# Autodesk Inventor assembly: AMR_Transm2
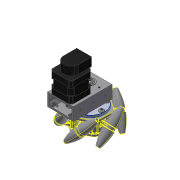
[picture p0: Inventor's stored thumbnail of the model, 180x180]
Saved by Autodesk Inventor 2018 (Build 220112000, 112)
## iProperties
Created: 2019-08-30
Part Number: AMR_Transm2
Document SubType Name: Assembly
Designer: Clevo
Author: Clevo
## Documents named in this file (20)
- E:\Hardware_Accelerated_Robot\Hardware\AMR_Transm2.iam
- E:\Hardware_Accelerated_Robot\Hardware\nema-17-12.snapshot.1\Nema 17\Nema 17.ipt
- E:\Hardware_Accelerated_Robot\Hardware\CustomParts\Transmission_Case.ipt
- E:\Hardware_Accelerated_Robot\Hardware\Bearings\7804K136_STAINLESS STEEL BALL BEARING.ipt
- E:\Hardware_Accelerated_Robot\Hardware\Wheels\am-3026L 4HD Mecanum Left V3 With Screws.ipt
- E:\Hardware_Accelerated_Robot\Hardware\Wheels\am-0096a 500 Hex Hub r2.ipt
- E:\Hardware_Accelerated_Robot\Hardware\CustomParts\Axle.ipt
- E:\Hardware_Accelerated_Robot\Hardware\Bearings\7804K147_STAINLESS STEEL BALL BEARING.ipt
- E:\Hardware_Accelerated_Robot\Hardware\Screws\94500A231_TYPE 316 SS BUTTON-HEAD SOCKET CAP SCREW.ipt
- E:\Hardware_Accelerated_Robot\Hardware\Screws\96660A215_FLANGED BUTTON-HEAD SOCKET CAP SCREW.ipt
- E:\Hardware_Accelerated_Robot\Hardware\Pulleys\gt2-40-teeth-bore-8mm-belt-6mm-1.snapshot.1\GT2_40T_8_6.ipt
- E:\Hardware_Accelerated_Robot\Hardware\Pulleys\timing-pulley-gt2-20t-8mm-bore-1.snapshot.8\GT2_20T-sh8.ipt
- E:\Hardware_Accelerated_Robot\Hardware\Bearings\5905K348_STEEL NEEDLE-ROLLER BEARING.ipt
- E:\Hardware_Accelerated_Robot\Hardware\AMR_Transm\Design Accelerator\Synchronous Belts Transmission1.iam
- E:\Hardware_Accelerated_Robot\Hardware\CustomParts\Tensioner.ipt
- E:\Hardware_Accelerated_Robot\Hardware\Screws\92137A262_CLASS 10.9 ALLOY STEEL BUTTON-HEAD CAP SCREW.ipt
- E:\Hardware_Accelerated_Robot\Hardware\Wheels\am-2538 - 4 in mecanum left wheel.ipt
- E:\Hardware_Accelerated_Robot\Hardware\Wheels\am-2256 4 in HiGrip Wheel.ipt
- E:\Hardware_Accelerated_Robot\Hardware\CustomParts\Transmission_Case_ForPrint.ipt
- E:\Hardware_Accelerated_Robot\Hardware\Screws\91385A211_THREAD-LOCKING CUP POINT SET SCREW.ipt
## Components (25 placed, 19 different names)
1. Nema 17:1 — Mate:1, Mate:2, Mate:3, Mate:4, Mate:32
2. Transmission_Case:1 — Mate:1, Mate:2, Mate:3, Mate:5, Mate:10, Mate:11, Mate:12, Mate:13, Mate:34, Mate:35, Mate:36, Flush:4, Flush:5, Mate:49
3. 7804K136_STAINLESS STEEL BALL BEARING:1 — Mate:4, Mate:5, Mate:33
4. am-3026L 4HD Mecanum Left V3 With Screws:1 — Mate:6, Mate:7, Mate:8
5. am-0096a 500 Hex Hub r2:1 — Mate:6, Mate:7, Mate:8, Mate:9, Flush:1, Angle:1, Mate:14, Mate:15, Mate:16, Mate:17, Mate:18, Mate:19, Mate:20, Mate:21, Mate:22, Mate:23, Mate:24, Mate:25, Mate:40, Mate:41, Mate:42, Mate:43, Mate:44, Mate:45, Mate:47
6. Axle:1 — Mate:9, Flush:1, Angle:1, Mate:26, Mate:28, Mate:29, Mate:30, Mate:48
7. 7804K147_STAINLESS STEEL BALL BEARING:1 — Mate:10, Mate:13, Mate:26
8. 7804K147_STAINLESS STEEL BALL BEARING:2 — Mate:11, Mate:12, Mate:27
9. 94500A231_TYPE 316 SS BUTTON-HEAD SOCKET CAP SCREW:1 — Mate:16, Mate:21
10. 94500A231_TYPE 316 SS BUTTON-HEAD SOCKET CAP SCREW:2 — Mate:17, Mate:22
11. 94500A231_TYPE 316 SS BUTTON-HEAD SOCKET CAP SCREW:3 — Mate:15, Mate:23
12. 94500A231_TYPE 316 SS BUTTON-HEAD SOCKET CAP SCREW:4 — Mate:14, Mate:20
13. 94500A231_TYPE 316 SS BUTTON-HEAD SOCKET CAP SCREW:5 — Mate:19, Mate:24
14. 94500A231_TYPE 316 SS BUTTON-HEAD SOCKET CAP SCREW:6 — Mate:18, Mate:25
15. 96660A215_FLANGED BUTTON-HEAD SOCKET CAP SCREW:1 — Mate:28, Mate:29, Mate:27
16. GT2_40T_8_6:1 — Mate:30, Flush:2
17. GT2_20T-sh8:1 — Mate:32, Flush:2, Mate:33
18. 5905K348_STEEL NEEDLE-ROLLER BEARING:1 — Mate:34, Mate:37
19. Synchronous Belts Transmission:1 [sub-assembly]
20. Tensioner:1 — Mate:35, Mate:36, Mate:37, Mate:38, Mate:39
21. 92137A262_CLASS 10.9 ALLOY STEEL BUTTON-HEAD CAP SCREW:1 — Mate:38, Mate:39
22. am-2538 - 4 in mecanum left wheel:1 — Mate:40, Mate:41, Mate:42
23. am-2256 4 in HiGrip Wheel:1 — Mate:43, Mate:44, Mate:45
24. Transmission_Case_ForPrint:1 — Flush:4, Flush:5, Mate:49
25. 91385A211_THREAD-LOCKING CUP POINT SET SCREW:1 — Mate:47, Mate:48
## Relationships (52: Mate 47, Flush 4, Angle 1)
- Mate:1: Nema 17:1 ↔ Transmission_Case:1
- Mate:2: Nema 17:1 ↔ Transmission_Case:1
- Mate:3: Nema 17:1 ↔ Transmission_Case:1
- Mate:4: Nema 17:1 ↔ 7804K136_STAINLESS STEEL BALL BEARING:1
- Mate:5: Transmission_Case:1 ↔ 7804K136_STAINLESS STEEL BALL BEARING:1
- Mate:6: am-3026L 4HD Mecanum Left V3 With Screws:1 ↔ am-0096a 500 Hex Hub r2:1
- Mate:7: am-3026L 4HD Mecanum Left V3 With Screws:1 ↔ am-0096a 500 Hex Hub r2:1
- Mate:8: am-3026L 4HD Mecanum Left V3 With Screws:1 ↔ am-0096a 500 Hex Hub r2:1
- Mate:9: am-0096a 500 Hex Hub r2:1 ↔ Axle:1
- Flush:1: am-0096a 500 Hex Hub r2:1 ↔ Axle:1
- Angle:1 (0 deg): am-0096a 500 Hex Hub r2:1 ↔ Axle:1
- Mate:10: Transmission_Case:1 ↔ 7804K147_STAINLESS STEEL BALL BEARING:1
- Mate:11: Transmission_Case:1 ↔ 7804K147_STAINLESS STEEL BALL BEARING:2
- Mate:12: Transmission_Case:1 ↔ 7804K147_STAINLESS STEEL BALL BEARING:2
- Mate:13: Transmission_Case:1 ↔ 7804K147_STAINLESS STEEL BALL BEARING:1
- Mate:14: am-0096a 500 Hex Hub r2:1 ↔ 94500A231_TYPE 316 SS BUTTON-HEAD SOCKET CAP SCREW:4
- Mate:15: am-0096a 500 Hex Hub r2:1 ↔ 94500A231_TYPE 316 SS BUTTON-HEAD SOCKET CAP SCREW:3
- Mate:16: am-0096a 500 Hex Hub r2:1 ↔ 94500A231_TYPE 316 SS BUTTON-HEAD SOCKET CAP SCREW:1
- Mate:17: am-0096a 500 Hex Hub r2:1 ↔ 94500A231_TYPE 316 SS BUTTON-HEAD SOCKET CAP SCREW:2
- Mate:18: am-0096a 500 Hex Hub r2:1 ↔ 94500A231_TYPE 316 SS BUTTON-HEAD SOCKET CAP SCREW:6
- Mate:19: am-0096a 500 Hex Hub r2:1 ↔ 94500A231_TYPE 316 SS BUTTON-HEAD SOCKET CAP SCREW:5
- Mate:20: am-0096a 500 Hex Hub r2:1 ↔ 94500A231_TYPE 316 SS BUTTON-HEAD SOCKET CAP SCREW:4
- Mate:21: am-0096a 500 Hex Hub r2:1 ↔ 94500A231_TYPE 316 SS BUTTON-HEAD SOCKET CAP SCREW:1
- Mate:22: am-0096a 500 Hex Hub r2:1 ↔ 94500A231_TYPE 316 SS BUTTON-HEAD SOCKET CAP SCREW:2
- Mate:23: am-0096a 500 Hex Hub r2:1 ↔ 94500A231_TYPE 316 SS BUTTON-HEAD SOCKET CAP SCREW:3
- Mate:24: am-0096a 500 Hex Hub r2:1 ↔ 94500A231_TYPE 316 SS BUTTON-HEAD SOCKET CAP SCREW:5
- Mate:25: am-0096a 500 Hex Hub r2:1 ↔ 94500A231_TYPE 316 SS BUTTON-HEAD SOCKET CAP SCREW:6
- Mate:26: Axle:1 ↔ 7804K147_STAINLESS STEEL BALL BEARING:1
- Mate:27: 7804K147_STAINLESS STEEL BALL BEARING:2 ↔ 96660A215_FLANGED BUTTON-HEAD SOCKET CAP SCREW:1
- Mate:28: Axle:1 ↔ 96660A215_FLANGED BUTTON-HEAD SOCKET CAP SCREW:1
- Mate:29: Axle:1 ↔ 96660A215_FLANGED BUTTON-HEAD SOCKET CAP SCREW:1
- Mate:30: Axle:1 ↔ GT2_40T_8_6:1
- Mate:32: Nema 17:1 ↔ GT2_20T-sh8:1
- Flush:2: GT2_40T_8_6:1 ↔ GT2_20T-sh8:1
- Mate:33: 7804K136_STAINLESS STEEL BALL BEARING:1 ↔ GT2_20T-sh8:1
- Mate:34: Transmission_Case:1 ↔ 5905K348_STEEL NEEDLE-ROLLER BEARING:1
- Mate:35: Transmission_Case:1 ↔ Tensioner:1
- Mate:36: Transmission_Case:1 ↔ Tensioner:1
- Mate:37: 5905K348_STEEL NEEDLE-ROLLER BEARING:1 ↔ Tensioner:1
- Mate:38: Tensioner:1 ↔ 92137A262_CLASS 10.9 ALLOY STEEL BUTTON-HEAD CAP SCREW:1
- Mate:39: Tensioner:1 ↔ 92137A262_CLASS 10.9 ALLOY STEEL BUTTON-HEAD CAP SCREW:1
- Mate:40: am-0096a 500 Hex Hub r2:1 ↔ am-2538 - 4 in mecanum left wheel:1
- Mate:41: am-0096a 500 Hex Hub r2:1 ↔ am-2538 - 4 in mecanum left wheel:1
- Mate:42: am-0096a 500 Hex Hub r2:1 ↔ am-2538 - 4 in mecanum left wheel:1
- Mate:43: am-0096a 500 Hex Hub r2:1 ↔ am-2256 4 in HiGrip Wheel:1
- Mate:44: am-0096a 500 Hex Hub r2:1 ↔ am-2256 4 in HiGrip Wheel:1
- Mate:45: am-0096a 500 Hex Hub r2:1 ↔ am-2256 4 in HiGrip Wheel:1
- Flush:4: Transmission_Case:1 ↔ Transmission_Case_ForPrint:1
- Mate:47: am-0096a 500 Hex Hub r2:1 ↔ 91385A211_THREAD-LOCKING CUP POINT SET SCREW:1
- Mate:48: Axle:1 ↔ 91385A211_THREAD-LOCKING CUP POINT SET SCREW:1
- Flush:5: Transmission_Case:1 ↔ Transmission_Case_ForPrint:1
- Mate:49: Transmission_Case:1 ↔ Transmission_Case_ForPrint:1
